# Autodesk Inventor assembly: roller
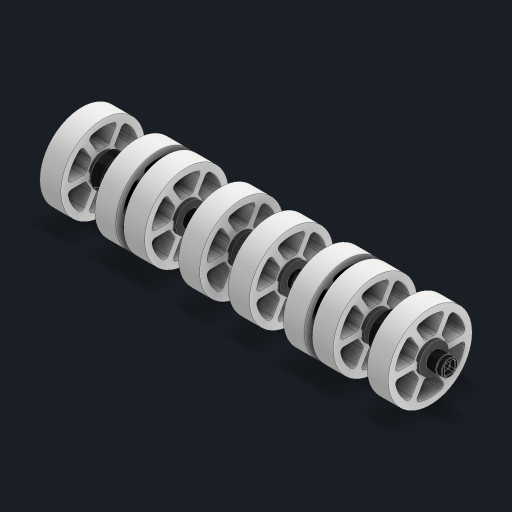
[picture p0: Inventor's stored thumbnail of the model, 512x512]
Saved by Autodesk Inventor 2024 (Build 280153000, 153)
## iProperties
Created: 2024-02-24
Part Number: roller
Document SubType Name: Assembly
Designer: Averey Ku
Author: Averey Ku
## Documents named in this file (9)
- D:\vex_robotics\hardware\cad\lil_zoom\intake\roller.iam
- D:\vex_robotics\hardware\cad\VEX-CAD-Inventor-1.41\Motion\Wheels\Flex Wheels\2.000 Flex Wheel\2.000 30A .500.ipt
- D:\vex_robotics\hardware\cad\VEX-CAD-Inventor-1.41\Motion\Wheels\Flex Wheels\2.000 Flex Wheel.ipt
- D:\vex_robotics\hardware\cad\VEX-CAD-Inventor-1.41\Motion\Wheels\Flex Wheels\VersaHex Adapters .125.ipt
- D:\vex_robotics\hardware\cad\VEX-CAD-Inventor-1.41\Motion\Shaft HS\HS Spacer\HSpacer .1250.ipt
- D:\vex_robotics\hardware\cad\VEX-CAD-Inventor-1.41\Motion\Shaft HS\HS Spacer.ipt
- D:\vex_robotics\hardware\cad\VEX-CAD-Inventor-1.41\Motion\Shaft HS\HS Spacer\HSpacer .2500.ipt
- D:\vex_robotics\hardware\cad\VEX-CAD-Inventor-1.41\Motion\Shaft HS\HS Spacer\HSpacer .5000.ipt
- D:\vex_robotics\hardware\cad\VEX-CAD-Inventor-1.41\Motion\Shaft HS\HS Shaft Collar.ipt
## Components (37 placed, 6 different names)
1. 2.000 30A .500:1
2. VersaHex Adapters .125:1 — Insert:2
3. VersaHex Adapters .125:2
4. 2.000 30A .500:2
5. VersaHex Adapters .125:3 — Insert:7
6. VersaHex Adapters .125:4
7. 2.000 30A .500:3
8. VersaHex Adapters .125:5
9. VersaHex Adapters .125:6 — Insert:12
10. 2.000 30A .500:4
11. VersaHex Adapters .125:7
12. VersaHex Adapters .125:8
13. 2.000 30A .500:5
14. VersaHex Adapters .125:9 — Insert:5
15. VersaHex Adapters .125:10
16. 2.000 30A .500:6
17. VersaHex Adapters .125:11 — Insert:13
18. VersaHex Adapters .125:12
19. 2.000 30A .500:7
20. VersaHex Adapters .125:13
21. VersaHex Adapters .125:14
22. 2.000 30A .500:8
23. VersaHex Adapters .125:15 — Insert:9
24. VersaHex Adapters .125:16 — Insert:4
25. HSpacer .1250:1 — Insert:1
26. HSpacer .2500:2 — Insert:1, Insert:2
27. HSpacer .5000:3 — Insert:5
28. HSpacer .1250:4
29. HSpacer .2500:5 — Insert:4
30. HS Shaft Collar:1 — Insert:6
31. HSpacer .1250:6 — Insert:6, Insert:7
32. HS Shaft Collar:3 — Insert:9
33. HSpacer .1250:7
34. HSpacer .5000:8 — Insert:10, Insert:13
35. HSpacer .1250:9 — Insert:10
36. HSpacer .5000:10 — Insert:12
37. HSpacer .1250:11
## Relationships (13: Insert 13)
- Insert:1: HSpacer .1250:1 ↔ HSpacer .2500:2
- Insert:2: VersaHex Adapters .125:1 ↔ HSpacer .2500:2
- [Insert]: HSpacer .1250:4 ↔ HSpacer .2500:5
- Insert:4: VersaHex Adapters .125:16 ↔ HSpacer .2500:5
- Insert:5: VersaHex Adapters .125:9 ↔ HSpacer .5000:3
- Insert:6: HS Shaft Collar:1 ↔ HSpacer .1250:6
- Insert:7: VersaHex Adapters .125:3 ↔ HSpacer .1250:6
- [Insert]: HS Shaft Collar:3 ↔ HSpacer .1250:7
- Insert:9: VersaHex Adapters .125:15 ↔ HS Shaft Collar:3
- Insert:10: HSpacer .5000:8 ↔ HSpacer .1250:9
- [Insert]: HSpacer .5000:10 ↔ HSpacer .1250:11
- Insert:12: VersaHex Adapters .125:6 ↔ HSpacer .5000:10
- Insert:13: VersaHex Adapters .125:11 ↔ HSpacer .5000:8
## Named parameters: d2_d0 = 0 mm, d7_d5 = 0 mm, d10_d9 = 0 mm
